# Autodesk Inventor assembly: z2cz
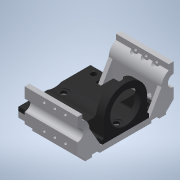
[picture p0: Inventor's stored thumbnail of the model, 180x180]
Saved by Autodesk Inventor 2020 (Build 240168000, 168)
## iProperties
Created: 2020-08-17
Part Number: z2cz
Material: Ogólny
Document SubType Name: Assembly
Designer: invin
Mass: 114.518 g
Surface Area: 435.452 cm^2
Volume: 96.74 cm^3
Density: 1.18377 g/cm^3
Author: invin
## Documents named in this file (3)
- D:\KONIECTEGOKOŁCHOZU\MGR\Model\Workspaces\Obszar roboczy\assembly_v3\Y\YSub2.iam
- D:\KONIECTEGOKOŁCHOZU\MGR\Model\Workspaces\Obszar roboczy\assembly_v3\Y\YFloatingMount.ipt
- D:\KONIECTEGOKOŁCHOZU\MGR\Model\Workspaces\Obszar roboczy\assembly_v3\Y\YRodMount.ipt
## Components (2 placed, 2 different names)
1. YFloatingMount:1 — Zestawiający:1, Zestawiający:2, Zestawiający:3
2. YRodMount:1 — Zestawiający:1, Zestawiający:2, Zestawiający:3
## Relationships (3: Mate 3)
- Zestawiający:1 [Mate]: YFloatingMount:1 ↔ YRodMount:1
- Zestawiający:2 [Mate]: YFloatingMount:1 ↔ YRodMount:1
- Zestawiający:3 [Mate]: YFloatingMount:1 ↔ YRodMount:1
